# Autodesk Inventor assembly: HexShaft+Toughbox-mini
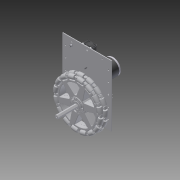
[picture p0: Inventor's stored thumbnail of the model, 180x180]
Saved by Autodesk Inventor 2013 (Build 170138000, 138)
## iProperties
Created: 2013-01-11
Part Number: HexShaft+Toughbox-mini
Document SubType Name: Assembly
Designer: Naphat
Translation Standard: STEP AP203
FileName: S:/Products/Gearboxes Spur Single Stage/Toughbox/Toughbox Mini/Toughbox-Mini.stp
PreProcessor: Unknown
PostProcessor: Build: 138, Release: 2013 RTM - Date: Thu 03/01/2012
Sent Units: millimeter
Uncertainty: 0.001
Author: Naphat
## Documents named in this file (22)
- C:\Users\carneeki\Desktop\Kiwi Robot\Drive Wheel\Drive Wheel.iam
- C:\Users\carneeki\Desktop\Kiwi Robot\Imported Components\Toughbox-mini\r6zz.ipt
- C:\Users\carneeki\Desktop\Kiwi Robot\Imported Components\Toughbox-mini\Toughbox_d07.ipt
- C:\Users\carneeki\Desktop\Kiwi Robot\Imported Components\Toughbox-mini\Toughbox_d05.ipt
- C:\Users\carneeki\Desktop\Kiwi Robot\Imported Components\Toughbox-mini\Toughbox_d08.ipt
- C:\Users\carneeki\Desktop\Kiwi Robot\Imported Components\Toughbox-mini\Toughbox_d06.ipt
- C:\Users\carneeki\Desktop\Kiwi Robot\Imported Components\Toughbox-mini\fr-6-zz.ipt
- C:\Users\carneeki\Desktop\Kiwi Robot\Imported Components\Toughbox-mini\fr-8-zz.ipt
- C:\Users\carneeki\Desktop\Kiwi Robot\Imported Components\Toughbox-mini\10-32_nylock_nut.ipt
- C:\Users\carneeki\Desktop\Kiwi Robot\Imported Components\Toughbox-mini\5-16_washer.ipt
- C:\Users\carneeki\Desktop\Kiwi Robot\Imported Components\Toughbox-mini\Toughbox_d09.ipt
- C:\Users\carneeki\Desktop\Kiwi Robot\Imported Components\Toughbox-mini\8mm_spring_clip.ipt
- C:\Users\carneeki\Desktop\Kiwi Robot\Imported Components\Toughbox-mini\Toughbox-mini_d01-5-12.ipt
- C:\Users\carneeki\Desktop\Kiwi Robot\Imported Components\Toughbox-mini\10-32x0625_shcs.ipt
- C:\Users\carneeki\Desktop\Kiwi Robot\Imported Components\Motors\CIM\CIM Motor.iam
- C:\Users\carneeki\Desktop\Kiwi Robot\Drive Wheel\CustomAM-2230.ipt
- C:\Users\carneeki\Desktop\Kiwi Robot\Imported Components\217-2613.20121203\217-2613.20121203.iam
- C:\Users\carneeki\Desktop\Kiwi Robot\Imported Components\217-2592.20121203.ipt
- C:\Users\carneeki\Desktop\Kiwi Robot\Imported Components\Hex Shaft.ipt
- C:\Users\carneeki\Desktop\Kiwi Robot\Imported Components\Victor884\Victor884.iam
- C:\Users\carneeki\Documents\Inventor\Content Center Files\R2013\en-US\ANSI B18.3(05)\ANSI B18.3 - 8-32 UNC - 1(31).ipt
- C:\Users\carneeki\Documents\Inventor\Content Center Files\R2013\en-US\IFI 100 107(2)\IFI 100_107 - No. 8 - 32 Top Insert Type.ipt
## Components (39 placed, 21 different names)
1. CIM Motor [sub-assembly]
2. CustomAM-2230:1 — Mate:10, Mate:11, Mate:19, Flush:2, Flush:3, Mate:21
3. 217-2613.20121203:1 [sub-assembly] — Insert:1, Insert:2, Mate:17, Mate:18
4. 217-2592.20121203:1 — Insert:2, Mate:17, Mate:18
5. 217-2592.20121203:2 — Mate:14, Mate:15, Mate:16, Insert:1
6. Hex Shaft:1 — Mate:12, Mate:13, Flush:1, Mate:14, Mate:15
7. Victor884:1 [sub-assembly] — Mate:19, Flush:2, Flush:3, Insert:3, Insert:4
8. Hexagon Socket Head Cap Screw - Inch No. 8 - 32 UNC - 1:1 — Insert:3, Mate:20
9. Hexagon Socket Head Cap Screw - Inch No. 8 - 32 UNC - 1:2 — Insert:4
10. Prevailing Torque Type Hex Nut - Inch (IFI) No. 8 - 32 Top Insert Type:1 — Mate:20, Mate:21
11. r6zz:1
12. r6zz:2 — Mate:9
13. Toughbox_d07:1
14. Toughbox_d05:1
15. Toughbox_d08:1
16. Toughbox_d06:1 — Mate:12, Mate:13
17. fr-6-zz:1 — Mate:10
18. fr-8-zz:1 — Mate:11, Mate:16
19. 10-32_nylock_nut:1
20. 10-32_nylock_nut:2
21. 10-32_nylock_nut:3
22. 10-32_nylock_nut:4
23. 5-16_washer:1
24. 5-16_washer:2
25. 5-16_washer:3
26. 5-16_washer:4
27. Toughbox_d09:1
28. Toughbox_d09:2
29. 8mm_spring_clip:1
30. 8mm_spring_clip:2
31. Toughbox-mini_d01-5-12:1 — Mate:9, Flush:1
32. 10-32x0625_shcs:1
33. 10-32x0625_shcs:2
34. 10-32x0625_shcs:3
35. 10-32x0625_shcs:4
36. 10-32x0625_shcs:5
37. 10-32x0625_shcs:6
38. 10-32x0625_shcs:7
39. 10-32x0625_shcs:8
## Relationships (20: Mate 13, Insert 4, Flush 3)
- Mate:9: r6zz:2 ↔ Toughbox-mini_d01-5-12:1
- Mate:10: CustomAM-2230:1 ↔ fr-6-zz:1
- Mate:11: CustomAM-2230:1 ↔ fr-8-zz:1
- Mate:12: Hex Shaft:1 ↔ Toughbox_d06:1
- Mate:13: Hex Shaft:1 ↔ Toughbox_d06:1
- Flush:1: Hex Shaft:1 ↔ Toughbox-mini_d01-5-12:1
- Mate:14: 217-2592.20121203:2 ↔ Hex Shaft:1
- Mate:15: 217-2592.20121203:2 ↔ Hex Shaft:1
- Mate:16 (2 mm): 217-2592.20121203:2 ↔ fr-8-zz:1
- Insert:1: 217-2613.20121203:1 ↔ 217-2592.20121203:2
- Insert:2: 217-2613.20121203:1 ↔ 217-2592.20121203:1
- Mate:17: 217-2613.20121203:1 ↔ 217-2592.20121203:1
- Mate:18: 217-2613.20121203:1 ↔ 217-2592.20121203:1
- Mate:19: CustomAM-2230:1 ↔ Victor884:1
- Flush:2 (25 mm): CustomAM-2230:1 ↔ Victor884:1
- Flush:3 (50 mm): CustomAM-2230:1 ↔ Victor884:1
- Mate:21: CustomAM-2230:1 ↔ Prevailing Torque Type Hex Nut - Inch (IFI) No. 8 - 32 Top Insert Type:1
- Insert:3: Victor884:1 ↔ Hexagon Socket Head Cap Screw - Inch No. 8 - 32 UNC - 1:1
- Insert:4: Victor884:1 ↔ Hexagon Socket Head Cap Screw - Inch No. 8 - 32 UNC - 1:2
- Mate:20: Hexagon Socket Head Cap Screw - Inch No. 8 - 32 UNC - 1:1 ↔ Prevailing Torque Type Hex Nut - Inch (IFI) No. 8 - 32 Top Insert Type:1
